# Autodesk Inventor assembly: dshape_fiber
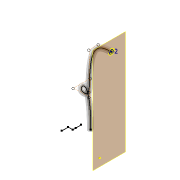
[picture p0: Inventor's stored thumbnail of the model, 180x180]
Saved by Autodesk Inventor 2019.4 (Build 234330000, 330)
## iProperties
Created: 2020-07-04
Part Number: dshape_fiber
Document SubType Name: Assembly
Designer: diederichbenedict
Author: diederichbenedict
## Documents named in this file (3)
- C:\Users\diederichbenedict\Dropbox\Dokumente\Promotion\PROJECTS\STORMoChip\GITHUB\CAD\Nanoscopy-on-the-cheap\Workspace\dshape_fiber.iam
- C:\Users\diederichbenedict\Dropbox\Dokumente\Promotion\PROJECTS\STORMoChip\GITHUB\CAD\Nanoscopy-on-the-cheap\Workspace\dshape_fiber_1.ipt
- C:\Users\diederichbenedict\Dropbox\Dokumente\Promotion\PROJECTS\STORMoChip\GITHUB\CAD\Nanoscopy-on-the-cheap\Workspace\dshape_fiber_2.ipt
## Components (2 placed, 2 different names)
1. dshape_fiber_1:1 — Insert:1
2. dshape_fiber_2:1 — Insert:1
## Relationships (1: Insert 1)
- Insert:1: dshape_fiber_1:1 ↔ dshape_fiber_2:1
